# Autodesk Inventor assembly: WolleyFan
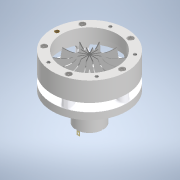
[picture p0: Inventor's stored thumbnail of the model, 180x180]
Saved by Autodesk Inventor 2021 (Build 250183000, 183)
## iProperties
Created: 2021-08-08
Part Number: WolleyFan
Document SubType Name: Assembly
Designer: Jack
Author: Jack
Title: Wolley Fan
## Documents named in this file (9)
- C:\Users\Jack\Projekt\Wolley\MEC_CentrifugalFan\CentrifugalFan.iam
- C:\Users\Jack\Projekt\Wolley\MEC_CentrifugalFan\Impeller.ipt
- C:\Users\Jack\Projekt\Wolley\MEC_CentrifugalFan\PCB.ipt
- C:\Users\Jack\Projekt\Wolley\MEC_CentrifugalFan\Spacer.ipt
- C:\Users\Jack\Projekt\Wolley\MEC_CentrifugalFan\Back.ipt
- C:\Users\Jack\Projekt\Wolley\MEC_CentrifugalFan\Front.ipt
- C:\Users\Jack\Projekt\Wolley\MEC_CentrifugalFan\M3ThreadedInsert.ipt
- C:\Users\Jack\Documents\Inventor\Content Center Files\R2021\en-US\DIN 912\DIN 912 - M3 x 0,5 x 30 x 18.ipt
- C:\Users\Jack\Projekt\Wolley\MEC_CentrifugalFan\Mabuchi_RS-385PV.ipt
## Components (21 placed, 8 different names)
1. Impeller:1
2. PCB:1 — Rotational:1, Rotational:2
3. Spacer:1
4. Back:1 — Rigid:6, Rigid:7, Rigid:8, Rigid:9, Rigid:10
5. Front:1 — Rigid:1, Rigid:2, Rigid:3, Rigid:4, Rigid:5, Insert:1, Insert:2, Insert:3, Insert:4, Insert:5
6. M3ThreadedInsert:1 — Rigid:1
7. M3ThreadedInsert:2 — Rigid:2
8. M3ThreadedInsert:3 — Rigid:3
9. M3ThreadedInsert:4 — Rigid:4
10. M3ThreadedInsert:5 — Rigid:5
11. M3ThreadedInsert:6 — Rigid:6
12. M3ThreadedInsert:7 — Rigid:9
13. M3ThreadedInsert:8 — Rigid:10
14. M3ThreadedInsert:9 — Rigid:8
15. M3ThreadedInsert:10 — Rigid:7
16. DIN 912 - replaced by DIN EN ISO 4762 M3 x 30:1 — Insert:1
17. DIN 912 - replaced by DIN EN ISO 4762 M3 x 30:2 — Insert:2
18. DIN 912 - replaced by DIN EN ISO 4762 M3 x 30:3 — Insert:3
19. DIN 912 - replaced by DIN EN ISO 4762 M3 x 30:4 — Insert:4
20. DIN 912 - replaced by DIN EN ISO 4762 M3 x 30:5 — Insert:5
21. Mabuchi_RS-385PV:1 — Rotational:1, Rotational:2
## Relationships (17: WeldJoint 10, Insert 5, RevoluteJoint 2)
- Rigid:1 [WeldJoint]: Front:1 ↔ M3ThreadedInsert:1
- Rigid:2 [WeldJoint]: Front:1 ↔ M3ThreadedInsert:2
- Rigid:3 [WeldJoint]: Front:1 ↔ M3ThreadedInsert:3
- Rigid:4 [WeldJoint]: Front:1 ↔ M3ThreadedInsert:4
- Rigid:5 [WeldJoint]: Front:1 ↔ M3ThreadedInsert:5
- Rigid:6 [WeldJoint]: Back:1 ↔ M3ThreadedInsert:6
- Rigid:7 [WeldJoint]: Back:1 ↔ M3ThreadedInsert:10
- Rigid:8 [WeldJoint]: Back:1 ↔ M3ThreadedInsert:9
- Rigid:9 [WeldJoint]: Back:1 ↔ M3ThreadedInsert:7
- Rigid:10 [WeldJoint]: Back:1 ↔ M3ThreadedInsert:8
- Insert:1: Front:1 ↔ DIN 912 - replaced by DIN EN ISO 4762 M3 x 30:1
- Insert:2: Front:1 ↔ DIN 912 - replaced by DIN EN ISO 4762 M3 x 30:2
- Insert:3: Front:1 ↔ DIN 912 - replaced by DIN EN ISO 4762 M3 x 30:3
- Insert:4: Front:1 ↔ DIN 912 - replaced by DIN EN ISO 4762 M3 x 30:4
- Insert:5: Front:1 ↔ DIN 912 - replaced by DIN EN ISO 4762 M3 x 30:5
- Rotational:1 [RevoluteJoint]: PCB:1 ↔ Mabuchi_RS-385PV:1
- Rotational:2 [RevoluteJoint]: PCB:1 ↔ Mabuchi_RS-385PV:1
